# Autodesk Inventor assembly: AssemblyAll
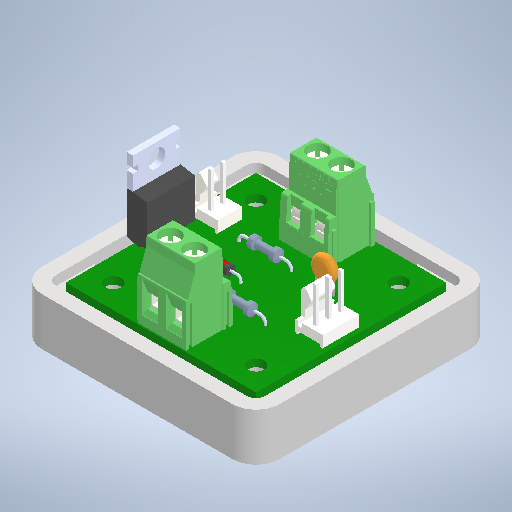
[picture p0: Inventor's stored thumbnail of the model, 512x512]
Saved by Autodesk Inventor 2025 (Build 290162010, 162A)
## iProperties
Created: 2025-11-03
Part Number: AssemblyAll
Document SubType Name: Assembly
Designer: João Vitor
Author: João Vitor
## Documents named in this file (3)
- C:\ProjectsOpenSource\SimpleAnalogDimmer\Inventor_Project\AssemblyAll.iam
- C:\ProjectsOpenSource\SimpleAnalogDimmer\Inventor_Project\LowerCase.ipt
- C:\ProjectsOpenSource\SimpleAnalogDimmer\Inventor_Project\PCB\DimmerCurso.iam
## Components (2 placed, 2 different names)
1. LowerCase:1 — Coincidente:1, Inserir:1, Coincidente:2
2. DimmerCurso:1 [sub-assembly] — Coincidente:1, Inserir:1, Coincidente:2
## Relationships (3: Mate 2, Insert 1)
- Coincidente:1 [Mate]: LowerCase:1 ↔ DimmerCurso:1
- Inserir:1: LowerCase:1 ↔ DimmerCurso:1
- Coincidente:2 [Mate]: LowerCase:1 ↔ DimmerCurso:1
